# Autodesk Inventor assembly: BRACKETS
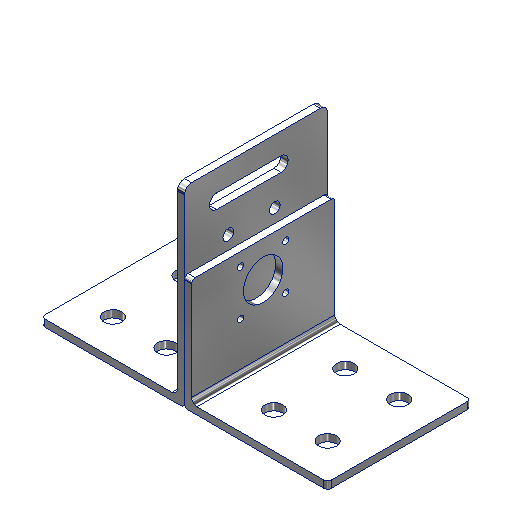
[picture p0: Inventor's stored thumbnail of the model, 512x512]
Saved by Autodesk Inventor 2025 (Build 290162000, 162)
## iProperties
Created: 2026-02-08
Part Number: BRACKETS
Document SubType Name: Assembly
Designer: HP
Author: HP
## Documents named in this file (3)
- C:\Users\HP\Desktop\TESIS 2\TFC2_20212123_MHinojosa\TFC2-20212123-HW\CAD\BRACKETS.iam
- C:\Users\HP\Desktop\TESIS 2\TFC2_20212123_MHinojosa\TFC2-20212123-HW\CAD\BRACKET_MOTOR.ipt
- C:\Users\HP\Desktop\TESIS 2\TFC2_20212123_MHinojosa\TFC2-20212123-HW\CAD\BRACKET_SENSOR.ipt
## Components (2 placed, 2 different names)
1. BRACKET_MOTOR:1 — Coincidencia:1, Nivelación:1, Nivelación:2
2. BRACKET_SENSOR:1 — Coincidencia:1, Nivelación:1, Nivelación:2
## Relationships (3: Flush 2, Mate 1)
- Coincidencia:1 [Mate]: BRACKET_MOTOR:1 ↔ BRACKET_SENSOR:1
- Nivelación:1 [Flush]: BRACKET_MOTOR:1 ↔ BRACKET_SENSOR:1
- Nivelación:2 [Flush]: BRACKET_MOTOR:1 ↔ BRACKET_SENSOR:1
